# Autodesk Inventor assembly: Assembly1
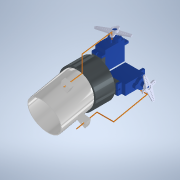
[picture p0: Inventor's stored thumbnail of the model, 180x180]
Saved by Autodesk Inventor 2021 (Build 250183000, 183)
## iProperties
Created: 2021-07-19
Part Number: Assembly1
Document SubType Name: Assembly
Designer: samlo
Author: samlo
## Documents named in this file (6)
- C:\Users\samlo\OneDrive\Documents\Assembly1.iam
- C:\Users\samlo\OneDrive\Documents\top tvc.ipt
- C:\Users\samlo\OneDrive\Documents\bottom tvc.ipt
- C:\Users\samlo\Downloads\servo-motor-sg90-7.snapshot.4\servorough_body.ipt
- C:\Users\samlo\Downloads\tower-pro-micro-servo-sg90-horn-1.snapshot.2\Tower pro micro servo SG90 HORN.ipt
- C:\Users\samlo\OneDrive\Documents\rod tvc.ipt
## Components (8 placed, 5 different names)
1. top tvc:1 — Ball:1, Rigid:1, Rigid:2
2. bottom tvc:1 — Ball:1, Cylindrical:1
3. servorough_body:1 — Rigid:2, Rotational:1
4. servorough_body:2 — Rigid:1, Rotational:2
5. Tower pro micro servo SG90 HORN:1 — Rotational:2, Rigid:3
6. Tower pro micro servo SG90 HORN:2 — Rotational:1, Cylindrical:5
7. rod tvc:1 — Rigid:3, Cylindrical:1
8. rod tvc:2 — Cylindrical:5
## Relationships (8: WeldJoint 3, RevoluteJoint 2, CylindricalJoint 2, BallJoint 1)
- Ball:1: top tvc:1 ↔ bottom tvc:1
- Rigid:1 [WeldJoint]: top tvc:1 ↔ servorough_body:2
- Rigid:2 [WeldJoint]: top tvc:1 ↔ servorough_body:1
- Rotational:1 [RevoluteJoint] (-7 mm): servorough_body:1 ↔ Tower pro micro servo SG90 HORN:2
- Rotational:2 [RevoluteJoint] (1 mm): servorough_body:2 ↔ Tower pro micro servo SG90 HORN:1
- Rigid:3 [WeldJoint]: Tower pro micro servo SG90 HORN:1 ↔ rod tvc:1
- Cylindrical:1: bottom tvc:1 ↔ rod tvc:1
- Cylindrical:5: Tower pro micro servo SG90 HORN:2 ↔ rod tvc:2
